# Autodesk Inventor assembly: Arm 1.1
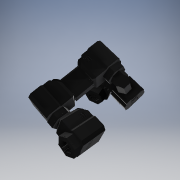
[picture p0: Inventor's stored thumbnail of the model, 180x180]
Saved by Autodesk Inventor 2017 SP1 (Build 210196100, 196)
## iProperties
Created: 2019-09-19
Part Number: Arm 1.1
Document SubType Name: Assembly
Designer: Dell
Author: Dell
## Documents named in this file (7)
- C:\Users\Zach\Documents\GitHub\tr2\Arm 1.1\Arm 1.1.iam
- C:\Users\Zach\Documents\GitHub\tr2\Arm 1.1\A01.ipt
- C:\Users\Zach\Documents\GitHub\tr2\Arm 1.1\A02.ipt
- C:\Users\Zach\Documents\GitHub\tr2\Actuator 2.0\XT-LG.iam
- C:\Users\Zach\Documents\GitHub\tr2\Actuator 2.0\XT-XL.iam
- C:\Users\Zach\Documents\GitHub\tr2\Actuator 2.0\XT-SM.iam
- C:\Users\Zach\Documents\GitHub\tr2\Arm 1.1\A03.ipt
## Components (10 placed, 6 different names)
1. XT-LG:1 [sub-assembly] — Mate:37, Mate:39, Mate:40, Mate:41, Mate:58, Mate:59
2. XT-LG:2 [sub-assembly] — Mate:48, Mate:49, Mate:50, Mate:51, Mate:60, Mate:61
3. XT-XL:1 [sub-assembly] — Mate:44, Mate:45, Mate:46, Mate:47, Mate:49, Mate:51
4. A01:1 — Mate:37, Mate:39, Mate:44, Mate:45, Mate:46, Mate:47, Mate:58, Mate:59, Mate:62, Mate:63, Mate:67, Mate:68
5. A02:1 — Mate:40, Mate:41, Mate:52, Mate:53
6. XT-SM:1 [sub-assembly] — Mate:52, Mate:53, Mate:54, Mate:55
7. XT-SM:2 [sub-assembly] — Mate:54, Mate:55, Mate:56, Mate:57
8. XT-SM:3 [sub-assembly] — Mate:56, Mate:57
9. XT-LG:3 [sub-assembly] — Mate:60, Mate:61, Mate:62, Mate:63
10. A03:1 — Mate:67, Mate:68
## Relationships (26: Mate 26)
- Mate:37: XT-LG:1 ↔ A01:1
- Mate:39: XT-LG:1 ↔ A01:1
- Mate:40: XT-LG:1 ↔ A02:1
- Mate:41: XT-LG:1 ↔ A02:1
- Mate:44: XT-XL:1 ↔ A01:1
- Mate:45: XT-XL:1 ↔ A01:1
- Mate:46: XT-XL:1 ↔ A01:1
- Mate:47: XT-XL:1 ↔ A01:1
- Mate:48: XT-LG:2
- Mate:49: XT-LG:2 ↔ XT-XL:1
- Mate:50: XT-LG:2
- Mate:51: XT-LG:2 ↔ XT-XL:1
- Mate:52: A02:1 ↔ XT-SM:1
- Mate:53: A02:1 ↔ XT-SM:1
- Mate:54: XT-SM:1 ↔ XT-SM:2
- Mate:55: XT-SM:1 ↔ XT-SM:2
- Mate:56: XT-SM:2 ↔ XT-SM:3
- Mate:57: XT-SM:2 ↔ XT-SM:3
- Mate:58: XT-LG:1 ↔ A01:1
- Mate:59: XT-LG:1 ↔ A01:1
- Mate:60: XT-LG:2 ↔ XT-LG:3
- Mate:61: XT-LG:2 ↔ XT-LG:3
- Mate:62: A01:1 ↔ XT-LG:3
- Mate:63: A01:1 ↔ XT-LG:3
- Mate:67: A01:1 ↔ A03:1
- Mate:68: A01:1 ↔ A03:1
